# Autodesk Inventor assembly: BaseAssembly
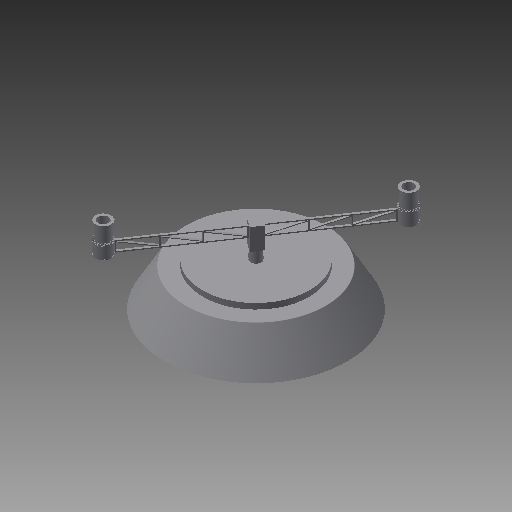
[picture p0: Inventor's stored thumbnail of the model, 512x512]
Saved by Autodesk Inventor 2018 (Build 220112000, 112)
## iProperties
Created: 2016-02-19
Part Number: BaseAssembly
Document SubType Name: Assembly
Designer: Tore Den Store
Author: Tore Den Store
## Documents named in this file (4)
- C:\Users\ToreDenStore\Documents\Inventor\Vertical axis wind turbine\BaseAssembly.iam
- C:\Users\ToreDenStore\Documents\Inventor\Vertical axis wind turbine\Main\MainBase.ipt
- C:\Users\ToreDenStore\Documents\Inventor\Vertical axis wind turbine\Main\Centre structure.ipt
- C:\Users\ToreDenStore\Documents\Inventor\Vertical axis wind turbine\WindPartRigid 1of2\Rigid holder.ipt
## Components (4 placed, 3 different names)
1. MainBase:1 — Mate:1, Mate:2, Rotational:1
2. Centre structure:1 — Rotational:1, Rigid:1, Rigid:2
3. Rigid holder:1 — Rigid:2
4. Rigid holder:2 — Rigid:1
## Relationships (5: Mate 2, WeldJoint 2, RevoluteJoint 1)
- Mate:1: MainBase:1
- Mate:2: MainBase:1
- Rotational:1 [RevoluteJoint]: MainBase:1 ↔ Centre structure:1
- Rigid:1 [WeldJoint]: Centre structure:1 ↔ Rigid holder:2
- Rigid:2 [WeldJoint]: Centre structure:1 ↔ Rigid holder:1
